# Autodesk Inventor assembly: Crank_Slider_Fixer
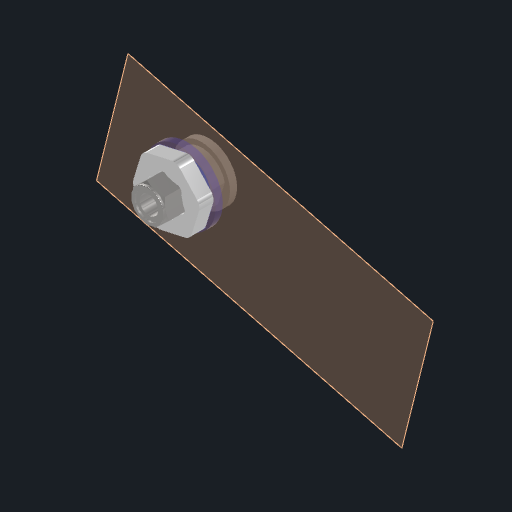
[picture p0: Inventor's stored thumbnail of the model, 512x512]
Saved by Autodesk Inventor 2024 (Build 280153000, 153)
## iProperties
Created: 2024-01-28
Part Number: Crank_Slider_Fixer
Document SubType Name: Assembly
Designer: 김대겸
Author: 김대겸
## Documents named in this file (6)
- C:\Users\ASUS\Desktop\Anti_Backlash_Structure_OP\MISUMI\Crank_Slider_Fixer.iam
- C:\Users\ASUS\Desktop\Anti_Backlash_Structure_OP\MISUMI\LED-0606.ipt
- C:\Users\ASUS\Desktop\Anti_Backlash_Structure_OP\v3_Frame\Ubber_Washer_1.5mm.ipt
- C:\Users\ASUS\Desktop\Anti_Backlash_Structure_OP\MISUMI\HNTL1N-ST-M4_203.ipt
- C:\Users\ASUS\Desktop\Anti_Backlash_Structure_OP\v3_Frame\Handmade tiered cover_9mm_Wide_ALU.ipt
- C:\Users\ASUS\Desktop\Anti_Backlash_Structure_OP\v3_Frame\Handmade tiered cover_9mm_Wide_ALU_Cover.ipt
## Components (5 placed, 5 different names)
1. LED-0606:1 — 메이트:6, 메이트:7, 각도:1
2. Ubber_Washer_1.5mm:1 — 메이트:6, 메이트:7, 삽입:2
3. HNTL1N-ST-M4_203:1 — 삽입:1, 메이트:12
4. Handmade tiered cover_9mm_Wide_ALU_Cover:2 — 메이트:9, 메이트:10, 메이트:11, 메이트:12, 각도:1
5. Handmade tiered cover_9mm_Wide_ALU:2 — 메이트:9, 메이트:10, 메이트:11, 삽입:1, 삽입:2
## Relationships (9: Mate 6, Insert 2, Angle 1)
- 메이트:6 [Mate] (3 mm): LED-0606:1 ↔ Ubber_Washer_1.5mm:1
- 메이트:7 [Mate]: LED-0606:1 ↔ Ubber_Washer_1.5mm:1
- 메이트:9 [Mate]: Handmade tiered cover_9mm_Wide_ALU_Cover:2 ↔ Handmade tiered cover_9mm_Wide_ALU:2
- 메이트:10 [Mate]: Handmade tiered cover_9mm_Wide_ALU_Cover:2 ↔ Handmade tiered cover_9mm_Wide_ALU:2
- 메이트:11 [Mate]: Handmade tiered cover_9mm_Wide_ALU_Cover:2 ↔ Handmade tiered cover_9mm_Wide_ALU:2
- 삽입:1 [Insert]: HNTL1N-ST-M4_203:1 ↔ Handmade tiered cover_9mm_Wide_ALU:2
- 삽입:2 [Insert]: Ubber_Washer_1.5mm:1 ↔ Handmade tiered cover_9mm_Wide_ALU:2
- 메이트:12 [Mate]: HNTL1N-ST-M4_203:1 ↔ Handmade tiered cover_9mm_Wide_ALU_Cover:2
- 각도:1 [Angle] (0 deg): LED-0606:1 ↔ Handmade tiered cover_9mm_Wide_ALU_Cover:2
